# Autodesk Inventor assembly: SERVO+GEARBOX ASSEMBLY
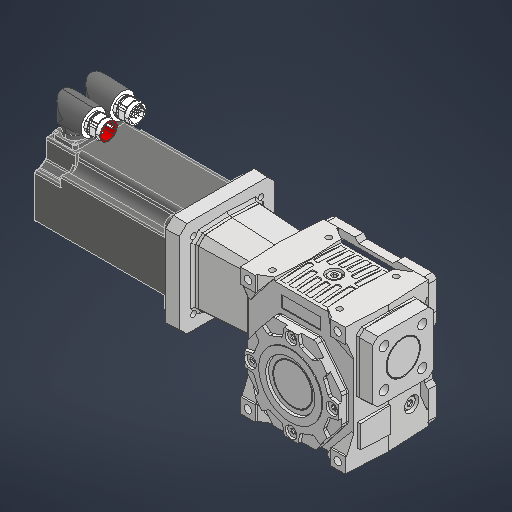
[picture p0: Inventor's stored thumbnail of the model, 512x512]
Saved by Autodesk Inventor 2025 (Build 290162000, 162)
## iProperties
Created: 2024-05-18
Part Number: SERVO+GEARBOX ASSEMBLY
Document SubType Name: Assembly
Designer: zulet
Author: zulet
## Documents named in this file (4)
- D:\UNAL\2024-1S\APM\Digital Factory\Packaging Machine\SERVO+GEARBOX ASSEMBLY.iam
- D:\UNAL\2024-1S\APM\Digital Factory\Worm Gear Boxes\148481481-9-dynabox_45_medium_p_h1_bm_f115-95_\dynabox_45_medium_p_h1_bm_f115-95_.iam
- D:\UNAL\2024-1S\APM\Digital Factory\Motors\148481278-9-servo_motor_mpl_b430p_mk72aa\servo_motor_mpl_b430p_mk72aa.iam
- D:\UNAL\2024-1S\APM\Digital Factory\Packaging Machine\Servo-Gear-MountingPlate.ipt
## Components (3 placed, 3 different names)
1. dynabox_45_medium_p_h1_bm_f115-95_:1 [sub-assembly] — Mate:1, Mate:2, Flush:1
2. servo_motor_mpl_b430p_mk72aa:1 [sub-assembly] — Mate:1, Mate:2
3. Servo-Gear-MountingPlate:1 — Flush:1
## Relationships (3: Mate 2, Flush 1)
- Mate:1: dynabox_45_medium_p_h1_bm_f115-95_:1 ↔ servo_motor_mpl_b430p_mk72aa:1
- Mate:2: dynabox_45_medium_p_h1_bm_f115-95_:1 ↔ servo_motor_mpl_b430p_mk72aa:1
- Flush:1: dynabox_45_medium_p_h1_bm_f115-95_:1 ↔ Servo-Gear-MountingPlate:1
